# Autodesk Inventor assembly: bmx_arm.v1
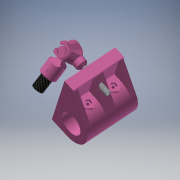
[picture p0: Inventor's stored thumbnail of the model, 180x180]
Saved by Autodesk Inventor 2016 (Build 200138000, 138)
## iProperties
Created: 2015-10-04
Part Number: bmx_arm.v1
Document SubType Name: Assembly
Designer: eedoga
Author: eedoga
## Documents named in this file (6)
- C:\Users\master\Documents\armstuff\bmx_arm.v1.iam
- C:\Users\master\Documents\!BMX_ARM\wrist-base1.ipt
- C:\Users\master\Documents\!BMX_ARM\wrist-forearm.ipt
- C:\Users\master\Documents\!BMX_ARM\carbon-fiber-forearm.ipt
- C:\Users\master\Documents\armstuff\pin.ipt
- C:\Users\master\Documents\armstuff\bike_gipper.ipt
## Components (5 placed, 5 different names)
1. wrist-base1:2 — Mate:4, Flush:12, Mate:6, Mate:7
2. wrist-forearm:2 — Mate:4, Flush:12, Flush:13, Mate:5, Angle:3, Flush:14
3. carbon-fiber-forearm:1 — Flush:13
4. pin:1 — Mate:6, Mate:7, Mate:8
5. bike_gipper:1 — Mate:8
## Relationships (9: Mate 5, Flush 3, Angle 1)
- Mate:4: wrist-base1:2 ↔ wrist-forearm:2
- Flush:12 (-0.1524 mm): wrist-base1:2 ↔ wrist-forearm:2
- Flush:13: wrist-forearm:2 ↔ carbon-fiber-forearm:1
- Mate:5: wrist-forearm:2
- Angle:3 (330 deg): wrist-forearm:2
- Flush:14: wrist-forearm:2
- Mate:6: wrist-base1:2 ↔ pin:1
- Mate:7: wrist-base1:2 ↔ pin:1
- Mate:8: pin:1 ↔ bike_gipper:1
